# Autodesk Inventor assembly: screw_sfnur02505t4dgc0-1100-p0_ss
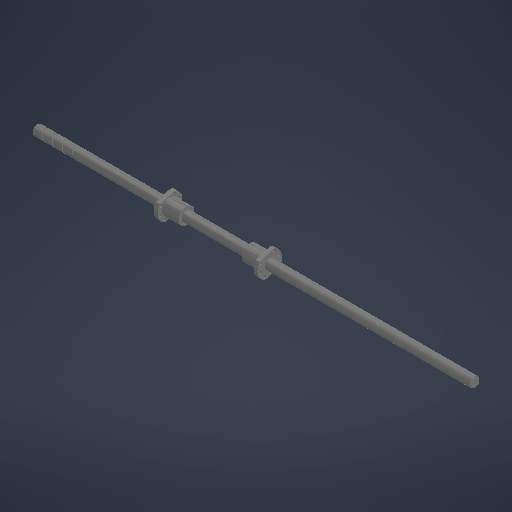
[picture p0: Inventor's stored thumbnail of the model, 512x512]
Saved by Autodesk Inventor 2025 (Build 290162000, 162)
## iProperties
Company: TraceParts S.A.
Created: 2024-05-18
Part Number: screw_sfnur02505t4dgc0-1100-p0_ss
Checked By: TraceParts S.A.
Catalog Web Link: www.traceparts.com
Document SubType Name: Assembly
Designer: TraceParts
Sending System: TraceParts v2
Major Version: 6.0
Minor Version: 0.0
Format Version: 0.0
Product Id: TraceParts v2
REFERENCE: SFNUR02505T4DGC0-1100-P0+SS
SUPPLIER: TBI MOTION TECHNOLOGY CO., LTD.
DESIGN: Ball Screw SFNUR02505T4DGC0-1100-P0+SS
TraceParts.PartNumber: 33-02092019-071003
TraceParts.PartTitle: Ball Screw / SFNU/SFU Series
TraceParts.InstanceId: 33-02092019-071003CY6VXZ7UBHK6J4ZSDJ9HBYK1A
TRACEPARTS: TRACEPARTS
TraceParts.PartLanguage: en
TraceParts.PartVersion: 1.1.3
Author: TraceParts
## Documents named in this file (3)
- D:\UNAL\2024-1S\APM\Digital Factory\Linear Guides & Ball Screws\screw_sfnur02505t4dgc0-1100-p0_ss.iam
- D:\UNAL\2024-1S\APM\Digital Factory\Linear Guides & Ball Screws\screw_sfnur02505t4dgc0-1100-p0_ss_01.ipt
- D:\UNAL\2024-1S\APM\Digital Factory\Linear Guides & Ball Screws\screw_sfnur02505t4dgc0-1100-p0_ss_02.ipt
## Components (3 placed, 3 different names)
1. screw_sfnur02505t4dgc0-1100-p0_ss_Temp_1:1 — Cylindrical:1
2. screw_sfnur02505t4dgc0-1100-p0_ss_Temp_2:1 — Cylindrical:1, Cylindrical:2
3. screw_sfnur02505t4dgc0-1100-p0_ss_01:2 — Cylindrical:2
## Relationships (2: CylindricalJoint 2)
- Cylindrical:1: screw_sfnur02505t4dgc0-1100-p0_ss_Temp_1:1 ↔ screw_sfnur02505t4dgc0-1100-p0_ss_Temp_2:1
- Cylindrical:2: screw_sfnur02505t4dgc0-1100-p0_ss_Temp_2:1 ↔ screw_sfnur02505t4dgc0-1100-p0_ss_01:2
